# Autodesk Inventor assembly: extruder
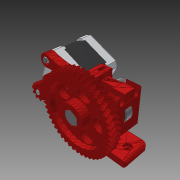
[picture p0: Inventor's stored thumbnail of the model, 180x180]
Saved by Autodesk Inventor 2014 (Build 180170000, 170)
## iProperties
Created: 2014-01-11
Part Number: extruder
Document SubType Name: Assembly
Designer: buben
Author: buben
## Documents named in this file (15)
- C:\Users\buben\Documents\GitHub\bacon\inventor files\assemblies\extruder.iam
- C:\Users\buben\Documents\GitHub\bacon\inventor files\3rd party components\gregs wade\jonaskuehling_gregs-wade-v3_jhead-BODY-ONLY.ipt
- C:\Users\buben\Documents\GitHub\bacon\inventor files\3rd party components\nema_17_stepper\Imported Components\NEMA 17\NEMA 17.iam
- C:\Users\buben\Documents\GitHub\bacon\inventor files\utils\washer_m3.ipt
- C:\Users\buben\Documents\Inventor\Content Center Files\R2014\en-US\ISO 4762(2)\ISO 4762 - M3 x 10ISO.ipt
- C:\Users\buben\Documents\GitHub\bacon\inventor files\3rd party components\bearing_608\Imported Components\608RS\608RS.ipt
- C:\Users\buben\Documents\GitHub\bacon\inventor files\3rd party components\gregs wade\smallgearmod_fixed.ipt
- C:\Users\buben\Documents\GitHub\bacon\inventor files\3rd party components\gregs wade\jonaskuehling_gregs-wade-v3_idler-only.ipt
- C:\Users\buben\Documents\GitHub\bacon\inventor files\3rd party components\gregs wade\biggearmod_fixed.ipt
- C:\Users\buben\Documents\Inventor\Content Center Files\R2014\en-US\ANSI B18.3.1M(6)\ANSI B18.3.1M - M3x0,5 x 35(1).ipt
- C:\Users\buben\Documents\GitHub\bacon\inventor files\utils\extruder_bearing_shaft.ipt
- C:\Users\buben\Documents\GitHub\bacon\inventor files\utils\washer_m8.ipt
- C:\Users\buben\Documents\Inventor\Content Center Files\R2014\en-US\CSN EN 24032\ISO 4032 - M8CSN EN.ipt
- C:\Users\buben\Documents\Inventor\Content Center Files\R2014\en-US\CSN EN 24014\ISO 4014 - M8 x 55CSN EN.ipt
- C:\Users\buben\Documents\Inventor\Content Center Files\R2014\en-US\ISO 7040\ISO 7040 - M3.ipt
## Components (26 placed, 14 different names)
1. jonaskuehling_gregs-wade-v3_jhead-BODY-ONLY:1 — Mate:1, Mate:2, Flush:1, Mate:3, Tangent:1, Tangent:2, Mate:4, Mate:5, Mate:6, Tangent:3, Tangent:4, Mate:10, Tangent:5, Tangent:6, Mate:11, Mate:13, Tangent:9, Tangent:10
2. NEMA 17:1 [sub-assembly] — Mate:3, Tangent:1, Tangent:2, Mate:7, Mate:8, Mate:9, Tangent:14, Tangent:15
3. CSN 02 1702 B B 3,2:1 — Mate:5, Insert:2
4. CSN 02 1702 B B 3,2:2 — Mate:4, Insert:1
5. CSN 02 1702 B B 3,2:3 — Mate:6, Insert:3
6. ISO 4762 M3 x 10:1 — Insert:1, Mate:7
7. ISO 4762 M3 x 10:2 — Insert:2, Mate:9
8. ISO 4762 M3 x 10:3 — Insert:3, Mate:8
9. 608RS:1 — Tangent:3, Tangent:4, Mate:10, Mate:25, Mate:26
10. 608RS:2 — Tangent:5, Tangent:6, Mate:11, Mate:27
11. Forged Socket Head Cap Screw - Metric M3x0,5 x 35:1 — Insert:4, Tangent:7, Tangent:8, Tangent:9, Tangent:10, Mate:34, Mate:36
12. smallgearmod_fixed:1 — Tangent:14, Tangent:15, Mate:37
13. jonaskuehling_gregs-wade-v3_idler-only:1 — Tangent:7, Tangent:8, Mate:12, Mate:13, Mate:15, Tangent:11, Tangent:12, Mate:16, Mate:33
14. biggearmod_fixed:1 — Mate:21, Mate:22, Tangent:13, Mate:24, Mate:37
15. CSN 02 1702 B B 3,2:4 — Insert:4, Mate:12
16. CSN 02 1702 B B 3,2:5 — Mate:33, Mate:34, Mate:35
17. extruder_bearing_shaft:1 — Mate:14, Mate:15, Tangent:11, Tangent:12
18. 608RS:3 — Mate:14, Mate:16
19. CSN 02 1702 B B 8,4:1 — Mate:17, Mate:18, Mate:19, Mate:20
20. CSN 02 1702 B B 8,4:2 — Mate:19, Mate:20, Mate:23, Mate:25
21. CSN 02 1702 B B 8,4:3 — Mate:17, Mate:18, Mate:24
22. CSN 02 1702 B B 8,4:4 — Mate:27, Mate:28, Mate:32
23. CSN EN 24014 M8 x 55:1 — Mate:21, Mate:22, Tangent:13, Mate:23, Mate:26, Mate:28, Mate:31
24. CSN EN 24032 M8:1 — Mate:29, Mate:30, Flush:2
25. CSN EN 24032 M8:2 — Mate:29, Mate:30, Flush:2, Mate:31, Mate:32
26. DIN EN ISO 7040 M3:1 — Mate:35, Mate:36
## Relationships (58: Mate 37, Tangent 15, Insert 4, Flush 2)
- Mate:1: jonaskuehling_gregs-wade-v3_jhead-BODY-ONLY:1
- Mate:2: jonaskuehling_gregs-wade-v3_jhead-BODY-ONLY:1
- Flush:1: jonaskuehling_gregs-wade-v3_jhead-BODY-ONLY:1
- Mate:3: jonaskuehling_gregs-wade-v3_jhead-BODY-ONLY:1 ↔ NEMA 17:1
- Tangent:1 (0.5 mm): jonaskuehling_gregs-wade-v3_jhead-BODY-ONLY:1 ↔ NEMA 17:1
- Tangent:2 (0.5 mm): jonaskuehling_gregs-wade-v3_jhead-BODY-ONLY:1 ↔ NEMA 17:1
- Mate:4: jonaskuehling_gregs-wade-v3_jhead-BODY-ONLY:1 ↔ CSN 02 1702 B B 3,2:2
- Mate:5: jonaskuehling_gregs-wade-v3_jhead-BODY-ONLY:1 ↔ CSN 02 1702 B B 3,2:1
- Mate:6: jonaskuehling_gregs-wade-v3_jhead-BODY-ONLY:1 ↔ CSN 02 1702 B B 3,2:3
- Insert:1: CSN 02 1702 B B 3,2:2 ↔ ISO 4762 M3 x 10:1
- Insert:2: CSN 02 1702 B B 3,2:1 ↔ ISO 4762 M3 x 10:2
- Insert:3: CSN 02 1702 B B 3,2:3 ↔ ISO 4762 M3 x 10:3
- Mate:7: NEMA 17:1 ↔ ISO 4762 M3 x 10:1
- Mate:8: NEMA 17:1 ↔ ISO 4762 M3 x 10:3
- Mate:9: NEMA 17:1 ↔ ISO 4762 M3 x 10:2
- Tangent:3: jonaskuehling_gregs-wade-v3_jhead-BODY-ONLY:1 ↔ 608RS:1
- Tangent:4: jonaskuehling_gregs-wade-v3_jhead-BODY-ONLY:1 ↔ 608RS:1
- Mate:10: jonaskuehling_gregs-wade-v3_jhead-BODY-ONLY:1 ↔ 608RS:1
- Tangent:5: jonaskuehling_gregs-wade-v3_jhead-BODY-ONLY:1 ↔ 608RS:2
- Tangent:6: jonaskuehling_gregs-wade-v3_jhead-BODY-ONLY:1 ↔ 608RS:2
- Mate:11: jonaskuehling_gregs-wade-v3_jhead-BODY-ONLY:1 ↔ 608RS:2
- Insert:4: Forged Socket Head Cap Screw - Metric M3x0,5 x 35:1 ↔ CSN 02 1702 B B 3,2:4
- Tangent:7: Forged Socket Head Cap Screw - Metric M3x0,5 x 35:1 ↔ jonaskuehling_gregs-wade-v3_idler-only:1
- Tangent:8: Forged Socket Head Cap Screw - Metric M3x0,5 x 35:1 ↔ jonaskuehling_gregs-wade-v3_idler-only:1
- Mate:12: jonaskuehling_gregs-wade-v3_idler-only:1 ↔ CSN 02 1702 B B 3,2:4
- Mate:13: jonaskuehling_gregs-wade-v3_jhead-BODY-ONLY:1 ↔ jonaskuehling_gregs-wade-v3_idler-only:1
- Tangent:9: jonaskuehling_gregs-wade-v3_jhead-BODY-ONLY:1 ↔ Forged Socket Head Cap Screw - Metric M3x0,5 x 35:1
- Tangent:10: jonaskuehling_gregs-wade-v3_jhead-BODY-ONLY:1 ↔ Forged Socket Head Cap Screw - Metric M3x0,5 x 35:1
- Mate:14: extruder_bearing_shaft:1 ↔ 608RS:3
- Mate:15: jonaskuehling_gregs-wade-v3_idler-only:1 ↔ extruder_bearing_shaft:1
- Tangent:11: jonaskuehling_gregs-wade-v3_idler-only:1 ↔ extruder_bearing_shaft:1
- Tangent:12: jonaskuehling_gregs-wade-v3_idler-only:1 ↔ extruder_bearing_shaft:1
- Mate:16: jonaskuehling_gregs-wade-v3_idler-only:1 ↔ 608RS:3
- Mate:17: CSN 02 1702 B B 8,4:1 ↔ CSN 02 1702 B B 8,4:3
- Mate:18: CSN 02 1702 B B 8,4:1 ↔ CSN 02 1702 B B 8,4:3
- Mate:19: CSN 02 1702 B B 8,4:1 ↔ CSN 02 1702 B B 8,4:2
- Mate:20: CSN 02 1702 B B 8,4:1 ↔ CSN 02 1702 B B 8,4:2
- Mate:21: biggearmod_fixed:1 ↔ CSN EN 24014 M8 x 55:1
- Mate:22: biggearmod_fixed:1 ↔ CSN EN 24014 M8 x 55:1
- Tangent:13 (0.5 mm): biggearmod_fixed:1 ↔ CSN EN 24014 M8 x 55:1
- Mate:23: CSN 02 1702 B B 8,4:2 ↔ CSN EN 24014 M8 x 55:1
- Mate:24: biggearmod_fixed:1 ↔ CSN 02 1702 B B 8,4:3
- Mate:25: 608RS:1 ↔ CSN 02 1702 B B 8,4:2
- Mate:26: 608RS:1 ↔ CSN EN 24014 M8 x 55:1
- Mate:27: 608RS:2 ↔ CSN 02 1702 B B 8,4:4
- Mate:28: CSN 02 1702 B B 8,4:4 ↔ CSN EN 24014 M8 x 55:1
- Mate:29: CSN EN 24032 M8:1 ↔ CSN EN 24032 M8:2
- Mate:30: CSN EN 24032 M8:1 ↔ CSN EN 24032 M8:2
- Flush:2: CSN EN 24032 M8:1 ↔ CSN EN 24032 M8:2
- Mate:31: CSN EN 24014 M8 x 55:1 ↔ CSN EN 24032 M8:2
- Mate:32: CSN 02 1702 B B 8,4:4 ↔ CSN EN 24032 M8:2
- Mate:33: jonaskuehling_gregs-wade-v3_idler-only:1 ↔ CSN 02 1702 B B 3,2:5
- Mate:34: Forged Socket Head Cap Screw - Metric M3x0,5 x 35:1 ↔ CSN 02 1702 B B 3,2:5
- Mate:35: CSN 02 1702 B B 3,2:5 ↔ DIN EN ISO 7040 M3:1
- Mate:36: Forged Socket Head Cap Screw - Metric M3x0,5 x 35:1 ↔ DIN EN ISO 7040 M3:1
- Tangent:14: NEMA 17:1 ↔ smallgearmod_fixed:1
- Tangent:15: NEMA 17:1 ↔ smallgearmod_fixed:1
- Mate:37 (1 mm): smallgearmod_fixed:1 ↔ biggearmod_fixed:1
